# Autodesk Inventor assembly: EVOTest
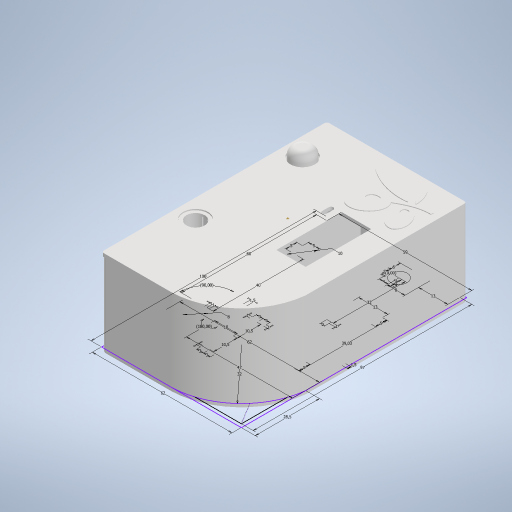
[picture p0: Inventor's stored thumbnail of the model, 512x512]
Saved by Autodesk Inventor 2023.2 (Build 272271000, 271)
## iProperties
Created: 2022-12-22
Part Number: EVOTest
Document SubType Name: Assembly
Designer: silvi
Author: silvi
## Documents named in this file (4)
- I:\Download\EVOTest\3D Model\EVOTest.iam
- I:\Download\EVOTest\3D Model\EvoTest_body_bottom_closed.ipt
- I:\Download\EVOTest\3D Model\EvoTest_top.ipt
- I:\Download\EVOTest\3D Model\EvoTest_button.ipt
## Components (3 placed, 3 different names)
1. EvoTest_body_bottom_closed:1 — Rigido:1
2. EvoTest_top:1 — Rigido:1, Inserimento:1, Cilindrico:1
3. EvoTest_button:1 — Inserimento:1, Cilindrico:1
## Relationships (3: WeldJoint 1, Insert 1, CylindricalJoint 1)
- Rigido:1 [WeldJoint]: EvoTest_body_bottom_closed:1 ↔ EvoTest_top:1
- Inserimento:1 (-1 mm): EvoTest_top:1 ↔ EvoTest_button:1
- Cilindrico:1 [CylindricalJoint]: EvoTest_top:1 ↔ EvoTest_button:1
